# Autodesk Inventor assembly: A
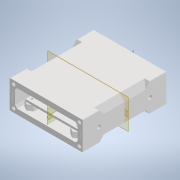
[picture p0: Inventor's stored thumbnail of the model, 180x180]
Saved by Autodesk Inventor 2022.2 (Build 262287000, 287)
## iProperties
Created: 2021-12-01
Part Number: A
Document SubType Name: Assembly
Designer: kfcs7
Author: kfcs7
## Documents named in this file (4)
- C:\Users\kfcs7\Desktop\Differential-Signal-Generator\models\A.iam
- C:\Users\kfcs7\Desktop\Differential-Signal-Generator\models\A-00.ipt
- C:\Users\kfcs7\Desktop\Differential-Signal-Generator\models\A-01.ipt
- C:\Users\kfcs7\Desktop\Differential-Signal-Generator\models\A-03.ipt
## Components (3 placed, 3 different names)
1. A-00:1 — Mate:1, Mate:2, Mate:3
2. A-01:1 — Mate:1, Mate:2, Mate:3, Rigid:1
3. A-03:1 — Rigid:1
## Relationships (4: Mate 3, WeldJoint 1)
- Mate:1: A-00:1 ↔ A-01:1
- Mate:2: A-00:1 ↔ A-01:1
- Mate:3: A-00:1 ↔ A-01:1
- Rigid:1 [WeldJoint]: A-01:1 ↔ A-03:1
